# Autodesk Inventor assembly: layout
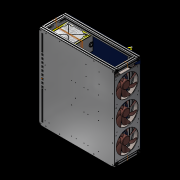
[picture p0: Inventor's stored thumbnail of the model, 180x180]
Saved by Autodesk Inventor 2018 (Build 220112000, 112)
## iProperties
Created: 2019-10-13
Part Number: layout
Material: 一般
Document SubType Name: Assembly
Designer: gisen
Author: gisen
## Documents named in this file (15)
- C:\Users\gisen\Documents\CAD\inventor\git\eatx_case\eatx_full\layout.iam
- C:\Users\gisen\Documents\CAD\inventor\git\eatx_case\eatx_full\resources\motherboard\Rampage V Extreme Assembly.iam
- C:\Users\gisen\Documents\CAD\inventor\git\eatx_case\eatx_full\resources\powersupply\ATX Power Supply v1.0.iam
- C:\Users\gisen\Documents\CAD\inventor\git\eatx_case\eatx_full\parts\backpanel.ipt
- C:\Users\gisen\Documents\CAD\inventor\git\eatx_case\eatx_full\parts\left_panel.ipt
- C:\Users\gisen\Documents\CAD\inventor\git\eatx_case\eatx_full\parts\right_panel.ipt
- C:\Users\gisen\Documents\CAD\inventor\git\eatx_case\eatx_full\resources\fan80\80x80x25 9 blade fan.iam
- C:\Users\gisen\Documents\CAD\inventor\git\eatx_case\eatx_full\parts\s450.ipt
- 00000010.ipt
- C:\Users\gisen\Documents\CAD\inventor\git\eatx_case\eatx_full\parts\s360.ipt
- C:\Users\gisen\Documents\CAD\inventor\git\eatx_case\eatx_full\parts\front_140mm.ipt
- C:\Users\gisen\Documents\CAD\inventor\git\eatx_case\eatx_full\parts\noctua14\Noctua NF-A14.iam
- C:\Users\gisen\Documents\CAD\inventor\git\eatx_case\eatx_full\parts\rtx3090\EVGA-FTW-3090.iam
- C:\Users\gisen\Documents\CAD\inventor\git\eatx_case\eatx_full\parts\s110.ipt
- C:\Users\gisen\Documents\CAD\inventor\git\eatx_case\eatx_full\parts\s440.ipt
## Components (25 placed, 10 different names)
1. Rampage V Extreme Assembly:1 [sub-assembly] — フラッシュ:136, メイト:140, フラッシュ:137, メイト:142, フラッシュ:139, メイト:172, メイト:173, メイト:174
2. ATX Power Supply v1.0:1 [sub-assembly] — メイト:143, メイト:144, フラッシュ:164
3. 00000010:35 — メイト:128, フラッシュ:72, 角度:2, 角度:3, フラッシュ:146, フラッシュ:149, フラッシュ:153, フラッシュ:157, フラッシュ:158, メイト:151, メイト:152, フラッシュ:161
4. 00000010:33 — メイト:129, フラッシュ:71, フラッシュ:72, 角度:1, 角度:2, フラッシュ:155, フラッシュ:156, フラッシュ:157, メイト:149, メイト:150, フラッシュ:161, メイト:157
5. 00000010:32 — メイト:40, フラッシュ:46, メイト:123, メイト:124, メイト:125, メイト:126, フラッシュ:70, フラッシュ:71, フラッシュ:132, 角度:1, メイト:142, フラッシュ:138, フラッシュ:139, フラッシュ:163, フラッシュ:156, メイト:148, メイト:154, フラッシュ:160
6. 00000010:41 — フラッシュ:141, フラッシュ:145, フラッシュ:148, フラッシュ:155, メイト:149, フラッシュ:159, メイト:171
7. 00000010:40 — フラッシュ:141, フラッシュ:145, フラッシュ:151, メイト:148
8. 00000010:43 — フラッシュ:142, フラッシュ:143, フラッシュ:146, フラッシュ:147, フラッシュ:153, メイト:152, メイト:153
9. 00000010:42 — フラッシュ:142, フラッシュ:143, フラッシュ:149, フラッシュ:150
10. 00000010:20 — フラッシュ:140, フラッシュ:144, フラッシュ:147, フラッシュ:148, メイト:150, メイト:151, メイト:157, フラッシュ:162
11. 00000010:21 — メイト:145, フラッシュ:140, フラッシュ:144, フラッシュ:150, フラッシュ:151, メイト:170
12. 00000010:26 — メイト:40, フラッシュ:46, フラッシュ:132, メイト:154, フラッシュ:159, フラッシュ:160
13. 00000010:34 — メイト:127, フラッシュ:70, 角度:3, フラッシュ:138, メイト:143, メイト:144, フラッシュ:164, フラッシュ:158, メイト:153, 角度:4, メイト:175
14. backpanel:1 — メイト:145, フラッシュ:163, メイト:155, メイト:156, メイト:175, メイト:176
15. left_panel:1 — メイト:123, メイト:124, メイト:128, メイト:129, メイト:130
16. right_panel:1 — メイト:125, メイト:126, メイト:127, メイト:130
17. 80x80x25 9 blade fan:1 [sub-assembly] — フラッシュ:134, フラッシュ:135, メイト:141, フラッシュ:136
18. 80x80x25 9 blade fan:2 [sub-assembly] — メイト:140, フラッシュ:134, フラッシュ:135, メイト:141, フラッシュ:137, メイト:176
19. ATX Power Supply v1.0:2 [sub-assembly] — メイト:155, 角度:4, メイト:156
20. front_140mm:1 — メイト:158, メイト:159, メイト:160, メイト:161, メイト:162, メイト:163, メイト:164, メイト:165, メイト:166, メイト:168, メイト:169, メイト:170, メイト:171, フラッシュ:162
21. front_140mm:2 — メイト:167, メイト:168, メイト:169
22. Noctua NF-A14:1 [sub-assembly] — メイト:158, メイト:159, メイト:160, メイト:167
23. Noctua NF-A14:2 [sub-assembly] — メイト:161, メイト:162, メイト:163
24. Noctua NF-A14:3 [sub-assembly] — メイト:164, メイト:165, メイト:166
25. EVGA-FTW-3090:1 [sub-assembly] — メイト:172, メイト:173, メイト:174
## Relationships (82: Mate 44, Flush 34, Angle 4)
- メイト:40 [Mate]: 00000010:32 ↔ 00000010:26
- フラッシュ:46 [Flush]: 00000010:32 ↔ 00000010:26
- メイト:123 [Mate]: 00000010:32 ↔ left_panel:1
- メイト:124 [Mate] (20 mm): 00000010:32 ↔ left_panel:1
- メイト:125 [Mate] (20 mm): 00000010:32 ↔ right_panel:1
- メイト:126 [Mate]: 00000010:32 ↔ right_panel:1
- メイト:127 [Mate]: 00000010:34 ↔ right_panel:1
- フラッシュ:70 [Flush]: 00000010:32 ↔ 00000010:34
- メイト:128 [Mate]: 00000010:35 ↔ left_panel:1
- メイト:129 [Mate]: 00000010:33 ↔ left_panel:1
- フラッシュ:71 [Flush]: 00000010:33 ↔ 00000010:32
- フラッシュ:72 [Flush]: 00000010:35 ↔ 00000010:33
- メイト:130 [Mate]: left_panel:1 ↔ right_panel:1
- フラッシュ:132 [Flush]: 00000010:32 ↔ 00000010:26
- 角度:1 [Angle] (180 deg): 00000010:33 ↔ 00000010:32
- 角度:2 [Angle] (180 deg): 00000010:35 ↔ 00000010:33
- 角度:3 [Angle] (180 deg): 00000010:35 ↔ 00000010:34
- メイト:140 [Mate] (41.73 mm): Rampage V Extreme Assembly:1 ↔ 80x80x25 9 blade fan:2
- フラッシュ:134 [Flush]: 80x80x25 9 blade fan:1 ↔ 80x80x25 9 blade fan:2
- フラッシュ:135 [Flush]: 80x80x25 9 blade fan:1 ↔ 80x80x25 9 blade fan:2
- メイト:141 [Mate] (3 mm): 80x80x25 9 blade fan:1 ↔ 80x80x25 9 blade fan:2
- フラッシュ:136 [Flush] (-1.402 mm): Rampage V Extreme Assembly:1 ↔ 80x80x25 9 blade fan:1
- フラッシュ:137 [Flush] (-8.035 mm): Rampage V Extreme Assembly:1 ↔ 80x80x25 9 blade fan:2
- メイト:142 [Mate] (5.602 mm): Rampage V Extreme Assembly:1 ↔ 00000010:32
- フラッシュ:138 [Flush]: 00000010:32 ↔ 00000010:34
- フラッシュ:139 [Flush] (-12 mm): Rampage V Extreme Assembly:1 ↔ 00000010:32
- メイト:143 [Mate] (8 mm): ATX Power Supply v1.0:1 ↔ 00000010:34
- メイト:144 [Mate] (3 mm): ATX Power Supply v1.0:1 ↔ 00000010:34
- メイト:145 [Mate]: 00000010:21 ↔ backpanel:1
- フラッシュ:163 [Flush]: 00000010:32 ↔ backpanel:1
- フラッシュ:164 [Flush]: ATX Power Supply v1.0:1 ↔ 00000010:34
- フラッシュ:140 [Flush]: 00000010:20 ↔ 00000010:21
- フラッシュ:141 [Flush]: 00000010:41 ↔ 00000010:40
- フラッシュ:142 [Flush]: 00000010:43 ↔ 00000010:42
- フラッシュ:143 [Flush]: 00000010:43 ↔ 00000010:42
- フラッシュ:144 [Flush]: 00000010:20 ↔ 00000010:21
- フラッシュ:145 [Flush]: 00000010:41 ↔ 00000010:40
- フラッシュ:146 [Flush] (20 mm): 00000010:35 ↔ 00000010:43
- フラッシュ:147 [Flush]: 00000010:43 ↔ 00000010:20
- フラッシュ:148 [Flush]: 00000010:41 ↔ 00000010:20
- フラッシュ:149 [Flush] (20 mm): 00000010:35 ↔ 00000010:42
- フラッシュ:150 [Flush]: 00000010:42 ↔ 00000010:21
- フラッシュ:151 [Flush]: 00000010:40 ↔ 00000010:21
- フラッシュ:153 [Flush]: 00000010:35 ↔ 00000010:43
- フラッシュ:155 [Flush]: 00000010:33 ↔ 00000010:41
- フラッシュ:156 [Flush]: 00000010:33 ↔ 00000010:32
- フラッシュ:157 [Flush]: 00000010:35 ↔ 00000010:33
- フラッシュ:158 [Flush]: 00000010:35 ↔ 00000010:34
- メイト:148 [Mate] (-20 mm): 00000010:32 ↔ 00000010:40
- メイト:149 [Mate] (-20 mm): 00000010:33 ↔ 00000010:41
- メイト:150 [Mate]: 00000010:33 ↔ 00000010:20
- メイト:151 [Mate]: 00000010:35 ↔ 00000010:20
- メイト:152 [Mate] (-20 mm): 00000010:35 ↔ 00000010:43
- メイト:153 [Mate] (-20 mm): 00000010:43 ↔ 00000010:34
- メイト:154 [Mate]: 00000010:32 ↔ 00000010:26
- フラッシュ:159 [Flush]: 00000010:41 ↔ 00000010:26
- フラッシュ:160 [Flush]: 00000010:32 ↔ 00000010:26
- メイト:155 [Mate]: backpanel:1 ↔ ATX Power Supply v1.0:2
- 角度:4 [Angle] (0 deg): 00000010:34 ↔ ATX Power Supply v1.0:2
- メイト:156 [Mate]: backpanel:1 ↔ ATX Power Supply v1.0:2
- フラッシュ:161 [Flush]: 00000010:35 ↔ 00000010:33
- メイト:157 [Mate] (15 mm): 00000010:33 ↔ 00000010:20
- メイト:158 [Mate]: front_140mm:1 ↔ Noctua NF-A14:1
- メイト:159 [Mate]: front_140mm:1 ↔ Noctua NF-A14:1
- メイト:160 [Mate]: front_140mm:1 ↔ Noctua NF-A14:1
- メイト:161 [Mate]: front_140mm:1 ↔ Noctua NF-A14:2
- メイト:162 [Mate]: front_140mm:1 ↔ Noctua NF-A14:2
- メイト:163 [Mate]: front_140mm:1 ↔ Noctua NF-A14:2
- メイト:164 [Mate]: front_140mm:1 ↔ Noctua NF-A14:3
- メイト:165 [Mate]: front_140mm:1 ↔ Noctua NF-A14:3
- メイト:166 [Mate]: front_140mm:1 ↔ Noctua NF-A14:3
- メイト:167 [Mate]: front_140mm:2 ↔ Noctua NF-A14:1
- メイト:168 [Mate]: front_140mm:1 ↔ front_140mm:2
- メイト:169 [Mate]: front_140mm:1 ↔ front_140mm:2
- メイト:170 [Mate]: 00000010:21 ↔ front_140mm:1
- メイト:171 [Mate]: 00000010:41 ↔ front_140mm:1
- フラッシュ:162 [Flush]: 00000010:20 ↔ front_140mm:1
- メイト:172 [Mate] (-0.4 mm): Rampage V Extreme Assembly:1 ↔ EVGA-FTW-3090:1
- メイト:173 [Mate]: Rampage V Extreme Assembly:1 ↔ EVGA-FTW-3090:1
- メイト:174 [Mate] (1 mm): Rampage V Extreme Assembly:1 ↔ EVGA-FTW-3090:1
- メイト:175 [Mate]: 00000010:34 ↔ backpanel:1
- メイト:176 [Mate]: backpanel:1 ↔ 80x80x25 9 blade fan:2
